# Autodesk Inventor assembly: Wash Chamber Assembly
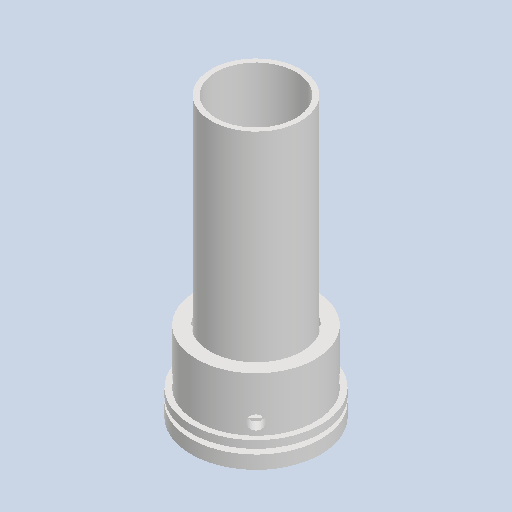
[picture p0: Inventor's stored thumbnail of the model, 512x512]
Saved by Autodesk Inventor 2024 (Build 280153000, 153)
## iProperties
Created: 2024-04-17
Part Number: Wash Chamber Assembly
Document SubType Name: Assembly
Designer: Tommy Rohmann
Author: Tommy Rohmann
## Documents named in this file (3)
- C:\Users\Tommy Rohmann\Documents\Repositories\Microgravity-Press-Washing-Machine\Sub-System Design and Documentation\3 Wash Chamber Assembly\Wash Chamber Assembly.iam
- C:\Users\Tommy Rohmann\Documents\Repositories\Microgravity-Press-Washing-Machine\Sub-System Design and Documentation\3 Wash Chamber Assembly\Wash Chamber Tube.ipt
- C:\Users\Tommy Rohmann\Documents\Repositories\Microgravity-Press-Washing-Machine\Sub-System Design and Documentation\3 Wash Chamber Assembly\Wash Chamber Conduit\Wash Chamber Conduit Assembly.iam
## Components (2 placed, 2 different names)
1. Wash Chamber Tube:1 — Mate:1, Mate:2
2. Wash Chamber Conduit Assembly:1 [sub-assembly] — Mate:1, Mate:2
## Relationships (2: Mate 2)
- Mate:1: Wash Chamber Tube:1 ↔ Wash Chamber Conduit Assembly:1
- Mate:2: Wash Chamber Tube:1 ↔ Wash Chamber Conduit Assembly:1
